# Autodesk Inventor assembly: MontagemDrone
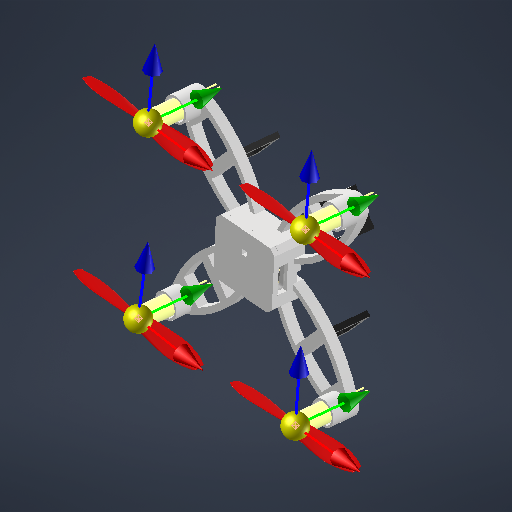
[picture p0: Inventor's stored thumbnail of the model, 512x512]
Saved by Autodesk Inventor 2027 (Build 310192000, 192)
## iProperties
Created: 2026-07-14
Part Number: MontagemDrone
Document SubType Name: Assembly
Designer: marcu
Mass: 15.1254 g
Surface Area: 211.381 cm^2
Volume: 13.9878 cm^3
Density: 1.08133 g/cm^3
Author: marcu
## iProperties of the stored document SKTAAAE010 v1.iam
Created: 2026-07-14
Part Number: SKTAAAE010 v1
Document SubType Name: Assembly
Designer: marcu
Mass: 0.0211812 g
Surface Area: 0.158648 cm^2
Volume: 0.00269824 cm^3
Density: 7.85 g/cm^3
Author: marcu
## iProperties of the stored document Peça58.ipt
Created: 2026-07-14
Part Number: Peça58
Material: Genérico
Document SubType Name: Modeling
Designer: marcu
Mass: 0.445404 g
Surface Area: 8.89255 cm^2
Volume: 0.445404 cm^3
Density: 1 g/cm^3
Appearance: Padrão
Author: marcu
## iProperties of the stored document U.FL-R-SMT-1_10_ v1.ipt
Created: 2026-07-14
Part Number: U.FL-R-SMT-1_10_ v1
Material: Stahl
Document SubType Name: Modeling
Designer: marcu
Mass: 0.0248383 g
Surface Area: 0.308242 cm^2
Volume: 0.00316412 cm^3
Density: 7.85 g/cm^3
Appearance: Padrão
Author: marcu
## iProperties of the stored document BOSS-EXTRUDE14_7_.ipt
Created: 2026-07-14
Part Number: BOSS-EXTRUDE14_7_
Material: Stahl
Document SubType Name: Modeling
Designer: marcu
Mass: 0.001413 g
Surface Area: 0.0216 cm^2
Volume: 0.00018 cm^3
Density: 7.85 g/cm^3
Appearance: Padrão
Author: marcu
## iProperties of the stored document BOSS-EXTRUDE14_1_.ipt
Created: 2026-07-14
Part Number: BOSS-EXTRUDE14_1_
Material: Stahl
Document SubType Name: Modeling
Designer: marcu
Mass: 0.0007065 g
Surface Area: 0.0138 cm^2
Volume: 9e-05 cm^3
Density: 7.85 g/cm^3
Appearance: Padrão
Author: marcu
## iProperties of the stored document BOSS-EXTRUDE14_2_.ipt
Created: 2026-07-14
Part Number: BOSS-EXTRUDE14_2_
Material: Stahl
Document SubType Name: Modeling
Designer: marcu
Mass: 0.001413 g
Surface Area: 0.0216 cm^2
Volume: 0.00018 cm^3
Density: 7.85 g/cm^3
Appearance: Padrão
Author: marcu
## iProperties of the stored document BOSS-EXTRUDE14_8_.ipt
Created: 2026-07-14
Part Number: BOSS-EXTRUDE14_8_
Material: Stahl
Document SubType Name: Modeling
Designer: marcu
Mass: 0.001413 g
Surface Area: 0.0216 cm^2
Volume: 0.00018 cm^3
Density: 7.85 g/cm^3
Appearance: Padrão
Author: marcu
## iProperties of the stored document BOSS-EXTRUDE7_7_.ipt
Created: 2026-07-14
Part Number: BOSS-EXTRUDE7_7_
Material: Stahl
Document SubType Name: Modeling
Designer: marcu
Mass: 0.00657054 g
Surface Area: 0.0816553 cm^2
Volume: 0.000837011 cm^3
Density: 7.85 g/cm^3
Appearance: Padrão
Author: marcu
## iProperties of the stored document CHAMFER9.ipt
Created: 2026-07-14
Part Number: CHAMFER9
Material: Stahl
Document SubType Name: Modeling
Designer: marcu
Mass: 0.324273 g
Surface Area: 3.04984 cm^2
Volume: 0.0413087 cm^3
Density: 7.85 g/cm^3
Appearance: Padrão
Author: marcu
## iProperties of the stored document BOSS-EXTRUDE14_6_.ipt
Created: 2026-07-14
Part Number: BOSS-EXTRUDE14_6_
Material: Stahl
Document SubType Name: Modeling
Designer: marcu
Mass: 0.001413 g
Surface Area: 0.0216 cm^2
Volume: 0.00018 cm^3
Density: 7.85 g/cm^3
Appearance: Padrão
Author: marcu
## iProperties of the stored document BOSS-EXTRUDE7_2_.ipt
Created: 2026-07-14
Part Number: BOSS-EXTRUDE7_2_
Material: Stahl
Document SubType Name: Modeling
Designer: marcu
Mass: 0.00657054 g
Surface Area: 0.0816553 cm^2
Volume: 0.000837011 cm^3
Density: 7.85 g/cm^3
Appearance: Padrão
Author: marcu
## iProperties of the stored document MIRROR2.ipt
Created: 2026-07-14
Part Number: MIRROR2
Material: Stahl
Document SubType Name: Modeling
Designer: marcu
Mass: 0.155659 g
Surface Area: 0.716778 cm^2
Volume: 0.0198292 cm^3
Density: 7.85 g/cm^3
Appearance: Padrão
Author: marcu
## iProperties of the stored document BOSS-EXTRUDE14_9_.ipt
Created: 2026-07-14
Part Number: BOSS-EXTRUDE14_9_
Material: Stahl
Document SubType Name: Modeling
Designer: marcu
Mass: 0.0007065 g
Surface Area: 0.0138 cm^2
Volume: 9e-05 cm^3
Density: 7.85 g/cm^3
Appearance: Padrão
Author: marcu
## iProperties of the stored document Peça60.ipt
Created: 2026-07-14
Part Number: Peça60
Material: Genérico
Document SubType Name: Modeling
Designer: marcu
Mass: 0.0113585 g
Surface Area: 2.54402 cm^2
Volume: 0.0113585 cm^3
Density: 1 g/cm^3
Appearance: Padrão
Author: marcu
## iProperties of the stored document BOSS-EXTRUDE7_9_.ipt
Created: 2026-07-14
Part Number: BOSS-EXTRUDE7_9_
Material: Stahl
Document SubType Name: Modeling
Designer: marcu
Mass: 0.00657054 g
Surface Area: 0.0816553 cm^2
Volume: 0.000837011 cm^3
Density: 7.85 g/cm^3
Appearance: Padrão
Author: marcu
## iProperties of the stored document BOSS-EXTRUDE7_5_.ipt
Created: 2026-07-14
Part Number: BOSS-EXTRUDE7_5_
Material: Stahl
Document SubType Name: Modeling
Designer: marcu
Mass: 0.00657054 g
Surface Area: 0.0816553 cm^2
Volume: 0.000837011 cm^3
Density: 7.85 g/cm^3
Appearance: Padrão
Author: marcu
## iProperties of the stored document XIAO-ESP32S3 v3 (1).iam
Created: 2025-02-17
Part Number: XIAO-ESP32S3 v2
Document SubType Name: Assembly
Designer: marcu
Mass: 1.76049 g
Surface Area: 22.0679 cm^2
Volume: 0.622843 cm^3
Density: 2.82654 g/cm^3
Title: XIAO-ESP32S3 v3.step
Sending System: Autodesk Translation Framework v13.20.0.188
Preprocessor: ST-DEVELOPER v20
## iProperties of the stored document BOSS-EXTRUDE7_8_.ipt
Created: 2026-07-14
Part Number: BOSS-EXTRUDE7_8_
Material: Stahl
Document SubType Name: Modeling
Designer: marcu
Mass: 0.00657054 g
Surface Area: 0.0816553 cm^2
Volume: 0.000837011 cm^3
Density: 7.85 g/cm^3
Appearance: Padrão
Author: marcu
## iProperties of the stored document USB TYPE C PORT.iam
Created: 2026-07-14
Part Number: USB TYPE C PORT
Document SubType Name: Assembly
Designer: marcu
Mass: 0.902663 g
Surface Area: 5.62653 cm^2
Volume: 0.114989 cm^3
Density: 7.85 g/cm^3
Author: marcu
## iProperties of the stored document USB TYPE C PORT (1).iam
Created: 2026-07-14
Part Number: USB TYPE C PORT (1)
Document SubType Name: Assembly
Designer: marcu
Mass: 0.902663 g
Surface Area: 5.62653 cm^2
Volume: 0.114989 cm^3
Density: 7.85 g/cm^3
Author: marcu
## iProperties of the stored document CUT-EXTRUDE5.ipt
Created: 2026-07-14
Part Number: CUT-EXTRUDE5
Material: Stahl
Document SubType Name: Modeling
Designer: marcu
Mass: 0.352291 g
Surface Area: 0.928211 cm^2
Volume: 0.0448779 cm^3
Density: 7.85 g/cm^3
Appearance: Padrão
Author: marcu
## iProperties of the stored document Seeed Studio XIAO-ESP32-S3 (Sense).iam
Created: 2026-07-14
Part Number: Seeed Studio XIAO-ESP32-S3 (Sense)
Document SubType Name: Assembly
Designer: marcu
Mass: 1.74913 g
Surface Area: 19.5239 cm^2
Volume: 0.611484 cm^3
Density: 2.86047 g/cm^3
Author: marcu
## iProperties of the stored document BOSS-EXTRUDE14_12_.ipt
Created: 2026-07-14
Part Number: BOSS-EXTRUDE14_12_
Material: Stahl
Document SubType Name: Modeling
Designer: marcu
Mass: 0.0007065 g
Surface Area: 0.0138 cm^2
Volume: 9e-05 cm^3
Density: 7.85 g/cm^3
Appearance: Padrão
Author: marcu
## iProperties of the stored document Pins.ipt
Created: 2026-07-14
Part Number: Pins
Material: Stahl
Document SubType Name: Modeling
Designer: marcu
Mass: 0.000607904 g
Surface Area: 0.022528 cm^2
Volume: 7.744e-05 cm^3
Density: 7.85 g/cm^3
Appearance: Padrão
Author: marcu
## iProperties of the stored document BOSS-EXTRUDE7_1_.ipt
Created: 2026-07-14
Part Number: BOSS-EXTRUDE7_1_
Material: Stahl
Document SubType Name: Modeling
Designer: marcu
Mass: 0.00657054 g
Surface Area: 0.0816553 cm^2
Volume: 0.000837011 cm^3
Density: 7.85 g/cm^3
Appearance: Padrão
Author: marcu
## iProperties of the stored document Shield.ipt
Created: 2026-07-14
Part Number: Shield
Material: Stahl
Document SubType Name: Modeling
Designer: marcu
Mass: 0.333866 g
Surface Area: 4.37924 cm^2
Volume: 0.0425307 cm^3
Density: 7.85 g/cm^3
Appearance: Padrão
Author: marcu
## iProperties of the stored document BOSS-EXTRUDE14_10_.ipt
Created: 2026-07-14
Part Number: BOSS-EXTRUDE14_10_
Material: Stahl
Document SubType Name: Modeling
Designer: marcu
Mass: 0.0007065 g
Surface Area: 0.0138 cm^2
Volume: 9e-05 cm^3
Density: 7.85 g/cm^3
Appearance: Padrão
Author: marcu
## iProperties of the stored document BOSS-EXTRUDE14_11_.ipt
Created: 2026-07-14
Part Number: BOSS-EXTRUDE14_11_
Material: Stahl
Document SubType Name: Modeling
Designer: marcu
Mass: 0.0007065 g
Surface Area: 0.0138 cm^2
Volume: 9e-05 cm^3
Density: 7.85 g/cm^3
Appearance: Padrão
Author: marcu
## iProperties of the stored document BOSS-EXTRUDE7_6_.ipt
Created: 2026-07-14
Part Number: BOSS-EXTRUDE7_6_
Material: Stahl
Document SubType Name: Modeling
Designer: marcu
Mass: 0.00657054 g
Surface Area: 0.0816553 cm^2
Volume: 0.000837011 cm^3
Density: 7.85 g/cm^3
Appearance: Padrão
Author: marcu
## iProperties of the stored document BOSS-EXTRUDE14_5_.ipt
Created: 2026-07-14
Part Number: BOSS-EXTRUDE14_5_
Material: Stahl
Document SubType Name: Modeling
Designer: marcu
Mass: 0.0007065 g
Surface Area: 0.0138 cm^2
Volume: 9e-05 cm^3
Density: 7.85 g/cm^3
Appearance: Padrão
Author: marcu
## iProperties of the stored document BOSS-EXTRUDE14_3_.ipt
Created: 2026-07-14
Part Number: BOSS-EXTRUDE14_3_
Material: Stahl
Document SubType Name: Modeling
Designer: marcu
Mass: 0.0007065 g
Surface Area: 0.0138 cm^2
Volume: 9e-05 cm^3
Density: 7.85 g/cm^3
Appearance: Padrão
Author: marcu
## iProperties of the stored document BOSS-EXTRUDE7_3_.ipt
Created: 2026-07-14
Part Number: BOSS-EXTRUDE7_3_
Material: Stahl
Document SubType Name: Modeling
Designer: marcu
Mass: 0.00657054 g
Surface Area: 0.0816553 cm^2
Volume: 0.000837011 cm^3
Density: 7.85 g/cm^3
Appearance: Padrão
Author: marcu
## iProperties of the stored document BOSS-EXTRUDE14_4_.ipt
Created: 2026-07-14
Part Number: BOSS-EXTRUDE14_4_
Material: Stahl
Document SubType Name: Modeling
Designer: marcu
Mass: 0.0007065 g
Surface Area: 0.0138 cm^2
Volume: 9e-05 cm^3
Density: 7.85 g/cm^3
Appearance: Padrão
Author: marcu
## iProperties of the stored document BOSS-EXTRUDE7_4_.ipt
Created: 2026-07-14
Part Number: BOSS-EXTRUDE7_4_
Material: Stahl
Document SubType Name: Modeling
Designer: marcu
Mass: 0.00657054 g
Surface Area: 0.0816553 cm^2
Volume: 0.000837011 cm^3
Density: 7.85 g/cm^3
Appearance: Padrão
Author: marcu
## iProperties of the stored document Body.ipt
Created: 2026-07-14
Part Number: Body
Material: Stahl
Document SubType Name: Modeling
Designer: marcu
Mass: 0.0205733 g
Surface Area: 0.13612 cm^2
Volume: 0.0026208 cm^3
Density: 7.85 g/cm^3
Appearance: Padrão
Author: marcu
## Documents named in this file (43)
- **C:\Users\marcu\Downloads\At Maker\MontagemDrone.iam*LocalDocs*xAaaaqmdaAaaaaaaaAaaaan1n0c*SKTAAAE010 v1.iam
- **C:\Users\marcu\Downloads\At Maker\MontagemDrone.iam*LocalDocs*xAaaaqzcaAaaaaaaaAaaaa014Ug*Body.ipt
- **C:\Users\marcu\Downloads\At Maker\MontagemDrone.iam*LocalDocs*xAaaaqtaaAaaaaaaaAaaaajlzYf*Pins.ipt
- **C:\Users\marcu\Downloads\At Maker\MontagemDrone.iam*LocalDocs*xAaaaazdaAaaaaaaaAaaaq4p2Cb*Peça58.ipt
- **C:\Users\marcu\Downloads\At Maker\MontagemDrone.iam*LocalDocs*xAaaaagdaAaaaaaaaAaaaanmj3g*U.FL-R-SMT-1_10_ v1.ipt
- **C:\Users\marcu\Downloads\At Maker\MontagemDrone.iam*LocalDocs*xAaaaaeaaAaaaaaaaAaaaqsylXa*BOSS-EXTRUDE14_7_.ipt
- **C:\Users\marcu\Downloads\At Maker\MontagemDrone.iam*LocalDocs*xAaaaa3caAaaaaaaaAaaaqxgzVc*BOSS-EXTRUDE14_1_.ipt
- **C:\Users\marcu\Downloads\At Maker\MontagemDrone.iam*LocalDocs*xAaaaa0caAaaaaaaaAaaaqy55Eb*BOSS-EXTRUDE14_2_.ipt
- **C:\Users\marcu\Downloads\At Maker\MontagemDrone.iam*LocalDocs*xAaaaa0caAaaaaaaaAaaaaij0Oc*BOSS-EXTRUDE14_8_.ipt
- **C:\Users\marcu\Downloads\At Maker\MontagemDrone.iam*LocalDocs*xAaaaabcaAaaaaaaaAaaaqd4qJd*BOSS-EXTRUDE7_7_.ipt
- **C:\Users\marcu\Downloads\At Maker\MontagemDrone.iam*LocalDocs*xAaaaaebaAaaaaaaaAaaaa33iZb*CHAMFER9.ipt
- **C:\Users\marcu\Downloads\At Maker\MontagemDrone.iam*LocalDocs*xAaaaamcaAaaaaaaaAaaaq3ycId*BOSS-EXTRUDE14_6_.ipt
- **C:\Users\marcu\Downloads\At Maker\MontagemDrone.iam*LocalDocs*xAaaaalcaAaaaaaaaAaaaaxdmWf*BOSS-EXTRUDE7_2_.ipt
- **C:\Users\marcu\Downloads\At Maker\MontagemDrone.iam*LocalDocs*xAaaaaxcaAaaaaaaaAaaaauz33g*MIRROR2.ipt
- **C:\Users\marcu\Downloads\At Maker\MontagemDrone.iam*LocalDocs*xAaaaandaAaaaaaaaAaaaqp5a3h*BOSS-EXTRUDE14_9_.ipt
- **C:\Users\marcu\Downloads\At Maker\MontagemDrone.iam*LocalDocs*xAaaaqdaaAaaaaaaaAaaaqq2xXb*Peça60.ipt
- **C:\Users\marcu\Downloads\At Maker\MontagemDrone.iam*LocalDocs*xAaaaqaaaAaaaaaaaAaaaqcnbLa*BOSS-EXTRUDE7_9_.ipt
- **C:\Users\marcu\Downloads\At Maker\MontagemDrone.iam*LocalDocs*xAaaaq1aaAaaaaaaaAaaaaeukHd*BOSS-EXTRUDE7_5_.ipt
- **C:\Users\marcu\Downloads\At Maker\MontagemDrone.iam*LocalDocs*xAaaaazdaAaaaaaaaAaaaqe15Xf*XIAO-ESP32S3 v3 (1).iam
- **C:\Users\marcu\Downloads\At Maker\MontagemDrone.iam*LocalDocs*xAaaaqdcaAaaaaaaaAaaaqzy4Xf*Seeed Studio XIAO-ESP32-S3 (Sense).iam
- **C:\Users\marcu\Downloads\At Maker\MontagemDrone.iam*LocalDocs*xAaaaqbaaAaaaaaaaAaaaqvkg2e*BOSS-EXTRUDE7_8_.ipt
- **C:\Users\marcu\Downloads\At Maker\MontagemDrone.iam*LocalDocs*xAaaaqbaaAaaaaaaaAaaaatz40c*USB TYPE C PORT.iam
- **C:\Users\marcu\Downloads\At Maker\MontagemDrone.iam*LocalDocs*xAaaaqhdaAaaaaaaaAaaaqvozSe*USB TYPE C PORT (1).iam
- **C:\Users\marcu\Downloads\At Maker\MontagemDrone.iam*LocalDocs*xAaaaqxdaAaaaaaaaAaaaa3osYd*BOSS-EXTRUDE7_4_.ipt
- **C:\Users\marcu\Downloads\At Maker\MontagemDrone.iam*LocalDocs*xAaaaqwcaAaaaaaaaAaaaa23gFb*BOSS-EXTRUDE7_3_.ipt
- **C:\Users\marcu\Downloads\At Maker\MontagemDrone.iam*LocalDocs*xAaaaqubaAaaaaaaaAaaaazybKh*BOSS-EXTRUDE14_4_.ipt
- **C:\Users\marcu\Downloads\At Maker\MontagemDrone.iam*LocalDocs*xAaaaqsdaAaaaaaaaAaaaqj33Ge*BOSS-EXTRUDE14_11_.ipt
- **C:\Users\marcu\Downloads\At Maker\MontagemDrone.iam*LocalDocs*xAaaaqzaaAaaaaaaaAaaaalubTg*BOSS-EXTRUDE14_3_.ipt
- **C:\Users\marcu\Downloads\At Maker\MontagemDrone.iam*LocalDocs*xAaaaqtdaAaaaaaaaAaaaqww4Za*BOSS-EXTRUDE14_5_.ipt
- **C:\Users\marcu\Downloads\At Maker\MontagemDrone.iam*LocalDocs*xAaaaqlaaAaaaaaaaAaaaa2tzTb*BOSS-EXTRUDE14_12_.ipt
- **C:\Users\marcu\Downloads\At Maker\MontagemDrone.iam*LocalDocs*xAaaaqqbaAaaaaaaaAaaaq2xaDb*BOSS-EXTRUDE7_1_.ipt
- **C:\Users\marcu\Downloads\At Maker\MontagemDrone.iam*LocalDocs*xAaaaqrbaAaaaaaaaAaaaqhx0Vf*BOSS-EXTRUDE14_10_.ipt
- **C:\Users\marcu\Downloads\At Maker\MontagemDrone.iam*LocalDocs*xAaaaqubaAaaaaaaaAaaaan2q0h*BOSS-EXTRUDE7_6_.ipt
- **C:\Users\marcu\Downloads\At Maker\MontagemDrone.iam*LocalDocs*xAaaaqddaAaaaaaaaAaaaqlpg5e*CUT-EXTRUDE5.ipt
- **C:\Users\marcu\Downloads\At Maker\MontagemDrone.iam*LocalDocs*xAaaaqnbaAaaaaaaaAaaaqterZf*Shield.ipt
- C:\Users\marcu\Downloads\At Maker\MontagemDrone.iam
- C:\Users\marcu\Downloads\At Maker\Frame1.ipt
- C:\Users\marcu\Downloads\At Maker\PCB.ipt
- C:\Users\marcu\Downloads\At Maker\TampaEletronica.ipt
- C:\Users\marcu\Downloads\At Maker\Trem_Pouso.ipt
- C:\Users\marcu\Downloads\At Maker\Motor.ipt
- C:\Users\marcu\Downloads\At Maker\Hélice1.ipt
- C:\Users\marcu\Downloads\XIAO-ESP32S3 v3 (1).step
## Components (16 placed, 7 different names)
1. Frame1:1 — Coincidente:1, Coincidente:2, Coincidente:4, Coincidente:5, Coincidente:6, Coincidente:7, Coincidente:8, Coincidente:9, Coincidente:10, Coincidente:11, Coincidente:12, Coincidente:13, Coincidente:14, Coincidente:15, Coincidente:16, Coincidente:17, Coincidente:18, Coincidente:19, Coincidente:20, Coincidente:21, Coincidente:22, Coincidente:23, Coincidente:24, Coincidente:25, Coincidente:26, Coincidente:27, Coincidente:29, Coincidente:30, Coincidente:31, Coincidente:32, Coincidente:33, Coincidente:34
2. PCB:1 — Coincidente:1, Coincidente:2, Coincidente:3, Coincidente:4
3. XIAO-ESP32S3 v3 (1):1 [sub-assembly] — Coincidente:3, Coincidente:5, Coincidente:6
4. TampaEletronica:1 — Coincidente:7, Coincidente:8, Coincidente:9
5. Trem_Pouso:1 — Coincidente:10, Coincidente:11, Coincidente:12, Coincidente:13, Coincidente:17, Coincidente:21
6. Trem_Pouso:2 — Coincidente:18, Coincidente:19, Coincidente:20
7. Trem_Pouso:3 — Coincidente:23, Coincidente:24, Coincidente:25
8. Trem_Pouso:4 — Coincidente:14, Coincidente:15, Coincidente:16, Coincidente:22
9. Motor:1 — Coincidente:32, Coincidente:33, Coincidente:35, Coincidente:36
10. Motor:2 — Coincidente:30, Coincidente:31, Coincidente:39, Coincidente:40
11. Motor:3 — Coincidente:26, Coincidente:27, Coincidente:37, Coincidente:38
12. Motor:4 — Coincidente:29, Coincidente:34, Coincidente:41, Coincidente:42
13. Hélice1:1 — Coincidente:37, Coincidente:38
14. Hélice1:2 — Coincidente:35, Coincidente:36
15. Hélice1:3 — Coincidente:41, Coincidente:42
16. Hélice1:4 — Coincidente:39, Coincidente:40
## Relationships (41: Mate 41)
- Coincidente:1 [Mate]: Frame1:1 ↔ PCB:1
- Coincidente:2 [Mate]: Frame1:1 ↔ PCB:1
- Coincidente:3 [Mate] (0.3 mm): PCB:1 ↔ XIAO-ESP32S3 v3 (1):1
- Coincidente:4 [Mate]: Frame1:1 ↔ PCB:1
- Coincidente:5 [Mate] (0.5 mm): Frame1:1 ↔ XIAO-ESP32S3 v3 (1):1
- Coincidente:6 [Mate] (0.5 mm): Frame1:1 ↔ XIAO-ESP32S3 v3 (1):1
- Coincidente:7 [Mate]: Frame1:1 ↔ TampaEletronica:1
- Coincidente:8 [Mate] (0.2 mm): Frame1:1 ↔ TampaEletronica:1
- Coincidente:9 [Mate] (0.2 mm): Frame1:1 ↔ TampaEletronica:1
- Coincidente:10 [Mate]: Frame1:1 ↔ Trem_Pouso:1
- Coincidente:11 [Mate]: Frame1:1 ↔ Trem_Pouso:1
- Coincidente:12 [Mate]: Frame1:1 ↔ Trem_Pouso:1
- Coincidente:13 [Mate] (13 mm): Frame1:1 ↔ Trem_Pouso:1
- Coincidente:14 [Mate]: Frame1:1 ↔ Trem_Pouso:4
- Coincidente:15 [Mate]: Frame1:1 ↔ Trem_Pouso:4
- Coincidente:16 [Mate]: Frame1:1 ↔ Trem_Pouso:4
- Coincidente:17 [Mate]: Frame1:1 ↔ Trem_Pouso:1
- Coincidente:18 [Mate]: Frame1:1 ↔ Trem_Pouso:2
- Coincidente:19 [Mate]: Frame1:1 ↔ Trem_Pouso:2
- Coincidente:20 [Mate]: Frame1:1 ↔ Trem_Pouso:2
- Coincidente:21 [Mate]: Frame1:1 ↔ Trem_Pouso:1
- Coincidente:22 [Mate]: Frame1:1 ↔ Trem_Pouso:4
- Coincidente:23 [Mate]: Frame1:1 ↔ Trem_Pouso:3
- Coincidente:24 [Mate]: Frame1:1 ↔ Trem_Pouso:3
- Coincidente:25 [Mate]: Frame1:1 ↔ Trem_Pouso:3
- Coincidente:26 [Mate]: Frame1:1 ↔ Motor:3
- Coincidente:27 [Mate]: Frame1:1 ↔ Motor:3
- Coincidente:29 [Mate]: Frame1:1 ↔ Motor:4
- Coincidente:30 [Mate]: Frame1:1 ↔ Motor:2
- Coincidente:31 [Mate]: Frame1:1 ↔ Motor:2
- Coincidente:32 [Mate]: Frame1:1 ↔ Motor:1
- Coincidente:33 [Mate]: Frame1:1 ↔ Motor:1
- Coincidente:34 [Mate]: Frame1:1 ↔ Motor:4
- Coincidente:35 [Mate]: Motor:1 ↔ Hélice1:2
- Coincidente:36 [Mate]: Motor:1 ↔ Hélice1:2
- Coincidente:37 [Mate]: Motor:3 ↔ Hélice1:1
- Coincidente:38 [Mate]: Motor:3 ↔ Hélice1:1
- Coincidente:39 [Mate]: Motor:2 ↔ Hélice1:4
- Coincidente:40 [Mate]: Motor:2 ↔ Hélice1:4
- Coincidente:41 [Mate]: Motor:4 ↔ Hélice1:3
- Coincidente:42 [Mate]: Motor:4 ↔ Hélice1:3
## Named parameters: Finish10_Area = 18.9295, Finish1_Area = 2.78875, Finish1_Thickness = 0.008 mm, Finish2_Area = 2.31685, Finish2_Thickness = 0.008 mm, Finish3_Area = 0.56, Finish4_Area = 0.995, Finish4_Thickness = 0.008 mm, Finish5_Area = 0.0415476, Finish6_Area = 0.124643, Finish7_Area = 0.16619, Finish8_Area = 14.1434, Finish8_Thickness = 0.008 mm, Finish9_Area = 14.1434, Finish9_Thickness = 0.008 mm
note: some values were not read from the file. Shown as the stored number, unit unknown: "Finish10_Area", "Finish1_Area", "Finish2_Area", "Finish3_Area", "Finish4_Area", "Finish5_Area", "Finish6_Area", "Finish7_Area", "Finish8_Area", "Finish9_Area".
